# Autodesk Inventor assembly: DStation
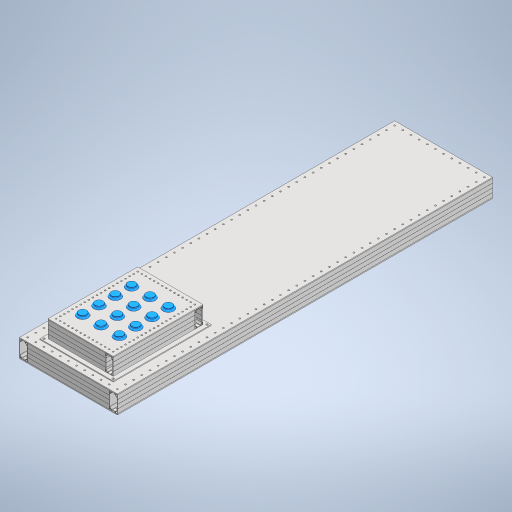
[picture p0: Inventor's stored thumbnail of the model, 512x512]
Saved by Autodesk Inventor 2023.4 (Build 274418000, 418)
## iProperties
Created: 2023-12-21
Part Number: DStation
Document SubType Name: Assembly
Designer: elija
Author: elija
## Documents named in this file (9)
- C:\Users\amrom\OneDrive\Desktop\Driver's station\DStation.iam
- C:\Users\elija\Downloads\BASE.ipt
- C:\Users\amrom\OneDrive\Desktop\Driver's station\REV MAXTUBE 10.ipt
- C:\Users\amrom\OneDrive\Desktop\Driver's station\REV 46 MAXTUBE.ipt
- C:\Users\elija\Downloads\joystick placeholder.ipt
- C:\Users\elija\Downloads\TOP DS.ipt
- C:\Users\amrom\OneDrive\Desktop\Driver's station\TOP DS new.ipt
- C:\Users\amrom\OneDrive\Desktop\Driver's station\BOTTOM DS new.ipt
- C:\Users\amrom\OneDrive\Desktop\Driver's station\Button Box\Button Box Assembly.iam
## Components (11 placed, 8 different names)
1. BASE:1 — Mate:1, Flush:1, Mate:2, Mate:3, Flush:2, Mate:4, Mate:5, Flush:3, Mate:6, Mate:7, Flush:4, Mate:8
2. REV MAXTUBE 10:1 — Mate:7, Flush:4, Mate:8, Flush:6, Flush:11, Flush:13
3. REV MAXTUBE 10:2 — Mate:3, Flush:2, Mate:4, Mate:42
4. REV 46 MAXTUBE:1 — Mate:5, Flush:3, Mate:6, Mate:15
5. REV 46 MAXTUBE:2 — Mate:1, Flush:1, Mate:2, Flush:7, Flush:8, Mate:14, Flush:9, Flush:10, Mate:43, Flush:12
6. joystick placeholder:1 — Flush:6, Flush:7, Mate:13, Mate:41
7. joystick placeholder:2 — Flush:8, Mate:13, Mate:40
8. TOP DS:1 — Mate:14, Flush:9, Mate:15, Mate:40, Mate:41
9. TOP DS new:1 — Mate:42, Flush:10, Flush:11, Mate:45, Mate:46
10. BOTTOM DS new:1 — Mate:43, Flush:12, Flush:13, Mate:44
11. Button Box Assembly:1 [sub-assembly] — Mate:44, Mate:45, Mate:46
## Relationships (30: Mate 18, Flush 12)
- Mate:1: BASE:1 ↔ REV 46 MAXTUBE:2
- Flush:1: BASE:1 ↔ REV 46 MAXTUBE:2
- Mate:2: BASE:1 ↔ REV 46 MAXTUBE:2
- Mate:3: BASE:1 ↔ REV MAXTUBE 10:2
- Flush:2: BASE:1 ↔ REV MAXTUBE 10:2
- Mate:4: BASE:1 ↔ REV MAXTUBE 10:2
- Mate:5: BASE:1 ↔ REV 46 MAXTUBE:1
- Flush:3: BASE:1 ↔ REV 46 MAXTUBE:1
- Mate:6: BASE:1 ↔ REV 46 MAXTUBE:1
- Mate:7: BASE:1 ↔ REV MAXTUBE 10:1
- Flush:4: BASE:1 ↔ REV MAXTUBE 10:1
- Mate:8: BASE:1 ↔ REV MAXTUBE 10:1
- Flush:6 (25.4 mm): REV MAXTUBE 10:1 ↔ joystick placeholder:1
- Flush:7 (25.4 mm): REV 46 MAXTUBE:2 ↔ joystick placeholder:1
- Flush:8 (-25.4 mm): REV 46 MAXTUBE:2 ↔ joystick placeholder:2
- Mate:13 (25.4 mm): joystick placeholder:1 ↔ joystick placeholder:2
- Mate:14: REV 46 MAXTUBE:2 ↔ TOP DS:1
- Flush:9: REV 46 MAXTUBE:2 ↔ TOP DS:1
- Mate:15: REV 46 MAXTUBE:1 ↔ TOP DS:1
- Mate:40: joystick placeholder:2 ↔ TOP DS:1
- Mate:41: joystick placeholder:1 ↔ TOP DS:1
- Mate:42: REV MAXTUBE 10:2 ↔ TOP DS new:1
- Flush:10: REV 46 MAXTUBE:2 ↔ TOP DS new:1
- Flush:11: REV MAXTUBE 10:1 ↔ TOP DS new:1
- Mate:43: REV 46 MAXTUBE:2 ↔ BOTTOM DS new:1
- Flush:12: REV 46 MAXTUBE:2 ↔ BOTTOM DS new:1
- Flush:13: REV MAXTUBE 10:1 ↔ BOTTOM DS new:1
- Mate:44: BOTTOM DS new:1 ↔ Button Box Assembly:1
- Mate:45: TOP DS new:1 ↔ Button Box Assembly:1
- Mate:46: TOP DS new:1 ↔ Button Box Assembly:1
